# Autodesk Inventor assembly: 08-20-2023-assieme con riduttore
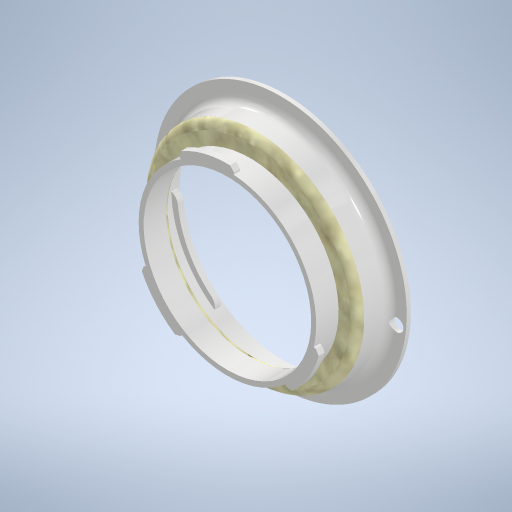
[picture p0: Inventor's stored thumbnail of the model, 512x512]
Saved by Autodesk Inventor 2023 (Build 270158000, 158)
## iProperties
Created: 2023-08-19
Part Number: 08-20-2023-assieme con riduttore
Document SubType Name: Assembly
Designer: Admin
Author: Admin
## Documents named in this file (4)
- C:\Users\Admin\Desktop\3DDDD\da stampanre\08-17-2023 adattatore cam dona\08-20-2023-assieme con riduttore.iam
- C:\Users\Admin\Desktop\3DDDD\da stampanre\08-17-2023 adattatore cam dona\CE2_adaptor_thin_2_v7.ipt
- C:\Users\Admin\Desktop\3DDDD\da stampanre\08-17-2023 adattatore cam dona\Sony_E-Mount_Body_Cap.ipt
- C:\Users\Admin\Desktop\3DDDD\da stampanre\08-17-2023 adattatore cam dona\riduttore.ipt
## Components (3 placed, 3 different names)
1. CE2_adaptor_thin_2_v7:1 — Coincidente:1
2. Sony_E-Mount_Body_Cap:1 — Coincidente:2
3. riduttore:1 — Coincidente:1, Coincidente:2
## Relationships (2: Mate 2)
- Coincidente:1 [Mate]: CE2_adaptor_thin_2_v7:1 ↔ riduttore:1
- Coincidente:2 [Mate]: Sony_E-Mount_Body_Cap:1 ↔ riduttore:1
